# Autodesk Inventor assembly: Press
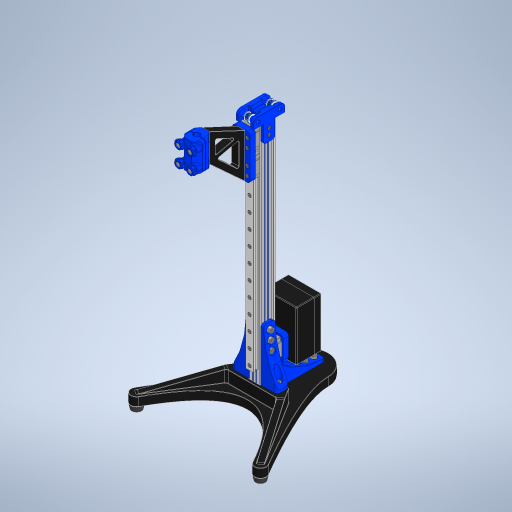
[picture p0: Inventor's stored thumbnail of the model, 512x512]
Saved by Autodesk Inventor 2024 (Build 280153000, 153)
## iProperties
Created: 2023-12-26
Part Number: Press
Document SubType Name: Assembly
Designer: denni
Author: denni
## Documents named in this file (28)
- D:\GIT\ThreadedInsertPress\Press.iam
- D:\GIT\ThreadedInsertPress\Parts\Others\AluminiumTSlotProfil20x20x420.ipt
- D:\GIT\ThreadedInsertPress\Parts\3D printed\PressBase.ipt
- D:\GIT\ThreadedInsertPress\Parts\Others\TS_04_12_364.ipt
- D:\Inventor\Content Center Files\R2024\de-DE\ISO 4762(1)\DIN EN ISO 4762 - M3 x 10.ipt
- D:\GIT\ThreadedInsertPress\Parts\3D printed\BraketBack.ipt
- D:\Inventor\Content Center Files\R2024\de-DE\ISO 4762(1)\DIN EN ISO 4762 - M5 x 16.ipt
- D:\Inventor\Content Center Files\R2024\de-DE\ISO 4762(1)\DIN EN ISO 4762 - M5 x 10.ipt
- D:\GIT\ThreadedInsertPress\Parts\3D printed\BraketSide.ipt
- D:\GIT\ThreadedInsertPress\Parts\Others\TW_04_12\TW_04_12.iam
- D:\GIT\ThreadedInsertPress\Parts\Others\RubberFeet\RubberFoot.iam
- D:\GIT\ThreadedInsertPress\Parts\3D printed\AdapterLinearGuideLong.ipt
- D:\Inventor\Content Center Files\R2024\de-DE\ISO 4762(1)\DIN EN ISO 4762 - M3 x 16.ipt
- D:\GIT\ThreadedInsertPress\Parts\3D printed\AdapterLinearGuideShort.ipt
- D:\GIT\ThreadedInsertPress\Parts\3D printed\IdlerBracket_Screws.ipt
- D:\GIT\ThreadedInsertPress\Parts\Others\Gt2TimingIdlerPulley16TW6B3\Gt2TimingIdlerPulley16TW6B3\Gt2TimingIdlerPulley16TW6B3.iam
- D:\GIT\ThreadedInsertPress\Parts\3D printed\IdlerBracket_Nuts.ipt
- D:\Inventor\Content Center Files\R2024\de-DE\ISO 4762(1)\DIN EN ISO 4762 - M3 x 6.ipt
- D:\Inventor\Content Center Files\R2024\de-DE\ISO 4762(1)\DIN EN ISO 4762 - M3 x 25.ipt
- D:\Inventor\Content Center Files\R2024\de-DE\ISO 4762(1)\DIN EN ISO 4762 - M5 x 20.ipt
- D:\GIT\ThreadedInsertPress\Parts\3D printed\ArmSolderingIron.ipt
- D:\GIT\ThreadedInsertPress\Parts\3D printed\BracketSolderingIron_1.ipt
- D:\Inventor\Content Center Files\R2024\de-DE\ISO 4762(1)\DIN EN ISO 4762 - M4 x 10.ipt
- D:\GIT\ThreadedInsertPress\Parts\3D printed\BracketSolderingIron_2.ipt
- D:\GIT\ThreadedInsertPress\Parts\3D printed\ScrewHead.ipt
- D:\Inventor\Content Center Files\R2024\de-DE\DIN EN ISO 4017\DIN EN ISO 4017 - M4 x 25.ipt
- D:\Inventor\Content Center Files\R2024\de-DE\DIN EN ISO 4032\DIN EN ISO 4032 - M3.ipt
- D:\GIT\ThreadedInsertPress\Parts\BatteryPack.iam
## Components (100 placed, 27 different names)
1. AluminiumTSlotProfil20x20x420:1 — Passend:1, Passend:2, Fluchtend:1, Fluchtend:2, Passend:3, Passend:4, Fluchtend:3, Fluchtend:4, Fluchtend:5, Passend:8, Passend:9, Fluchtend:6, Fluchtend:7, Passend:31, Passend:32, Passend:33, Fluchtend:8
2. PressBase:1 — Passend:1, Passend:2, Fluchtend:1, Passend:5, Passend:6, Passend:7, Passend:10, Passend:11, Passend:18, Passend:19, Passend:20, Passend:21, Passend:22, Passend:23
3. TS_04_12_364:1 — Fluchtend:2, Passend:3, Fluchtend:5, Einfügen:1, Einfügen:2, Einfügen:3, Einfügen:4, Einfügen:5, Einfügen:6, Einfügen:7, Einfügen:8, Einfügen:9, Einfügen:10, Einfügen:11, Einfügen:12, Einfügen:13, Einfügen:14, Einfügen:15, Passend:12, Passend:13, Passend:14, Passend:15
4. TS_04_12_364:2 — Passend:4, Fluchtend:3, Fluchtend:4, Einfügen:16, Einfügen:17, Einfügen:18, Einfügen:19, Einfügen:20, Einfügen:21, Einfügen:22, Einfügen:23, Einfügen:24, Einfügen:25, Einfügen:26, Einfügen:27, Einfügen:28, Einfügen:29, Einfügen:30, Passend:16, Passend:17
5. DIN EN ISO 4762 M3 x 10:1 — Einfügen:1
6. DIN EN ISO 4762 M3 x 10:2 — Einfügen:2
7. DIN EN ISO 4762 M3 x 10:3 — Einfügen:3
8. DIN EN ISO 4762 M3 x 10:4 — Einfügen:4
9. DIN EN ISO 4762 M3 x 10:5 — Einfügen:5
10. DIN EN ISO 4762 M3 x 10:6 — Einfügen:6
11. DIN EN ISO 4762 M3 x 10:7 — Einfügen:7
12. DIN EN ISO 4762 M3 x 10:8 — Einfügen:8
13. DIN EN ISO 4762 M3 x 10:9 — Einfügen:9
14. DIN EN ISO 4762 M3 x 10:10 — Einfügen:10
15. DIN EN ISO 4762 M3 x 10:11 — Einfügen:11
16. DIN EN ISO 4762 M3 x 10:12 — Einfügen:12
17. DIN EN ISO 4762 M3 x 10:13 — Einfügen:13
18. DIN EN ISO 4762 M3 x 10:14 — Einfügen:14
19. DIN EN ISO 4762 M3 x 10:15 — Einfügen:15
20. DIN EN ISO 4762 M3 x 10:16 — Einfügen:16
21. DIN EN ISO 4762 M3 x 10:17 — Einfügen:17
22. DIN EN ISO 4762 M3 x 10:18 — Einfügen:18
23. DIN EN ISO 4762 M3 x 10:19 — Einfügen:19
24. DIN EN ISO 4762 M3 x 10:20 — Einfügen:20
25. DIN EN ISO 4762 M3 x 10:21 — Einfügen:21
26. DIN EN ISO 4762 M3 x 10:22 — Einfügen:22
27. DIN EN ISO 4762 M3 x 10:23 — Einfügen:23
28. DIN EN ISO 4762 M3 x 10:24 — Einfügen:24
29. DIN EN ISO 4762 M3 x 10:25 — Einfügen:25
30. DIN EN ISO 4762 M3 x 10:26 — Einfügen:26
31. DIN EN ISO 4762 M3 x 10:27 — Einfügen:27
32. DIN EN ISO 4762 M3 x 10:28 — Einfügen:28
33. DIN EN ISO 4762 M3 x 10:29 — Einfügen:29
34. DIN EN ISO 4762 M3 x 10:30 — Einfügen:30
35. BraketBack:1 — Passend:5, Passend:6, Passend:7, Einfügen:31, Einfügen:32, Einfügen:33, Einfügen:34, Einfügen:35
36. DIN EN ISO 4762 M5 x 16:1 — Einfügen:31
37. DIN EN ISO 4762 M5 x 16:2 — Einfügen:32
38. DIN EN ISO 4762 M5 x 16:3 — Einfügen:33
39. DIN EN ISO 4762 M5 x 10:1 — Einfügen:34
40. DIN EN ISO 4762 M5 x 10:2 — Einfügen:35
41. BraketSide:1 — Passend:9, Passend:10, Fluchtend:6, Einfügen:36, Einfügen:37, Einfügen:38, Einfügen:39
42. BraketSide:2 — Passend:8, Passend:11, Fluchtend:7, Einfügen:40, Einfügen:41, Einfügen:42, Einfügen:43
43. DIN EN ISO 4762 M5 x 16:4 — Einfügen:36
44. DIN EN ISO 4762 M5 x 10:3 — Einfügen:37
45. DIN EN ISO 4762 M5 x 10:4 — Einfügen:38
46. DIN EN ISO 4762 M5 x 10:5 — Einfügen:39
47. DIN EN ISO 4762 M5 x 10:6 — Einfügen:40
48. DIN EN ISO 4762 M5 x 10:7 — Einfügen:41
49. DIN EN ISO 4762 M5 x 10:8 — Einfügen:42
50. DIN EN ISO 4762 M5 x 16:5 — Einfügen:43
51. TW_04_12:1 [sub-assembly] — Passend:13, Passend:15, Passend:24, Passend:25, Passend:26
52. TW_04_12:2 [sub-assembly] — Passend:12, Passend:14, Passend:24, Passend:27
53. TW_04_12:3 [sub-assembly] — Passend:16, Passend:17, Passend:28, Passend:29, Passend:30
54. RubberFoot:1 [sub-assembly] — Passend:18, Passend:22
55. RubberFoot:2 [sub-assembly] — Passend:19, Passend:21
56. RubberFoot:3 [sub-assembly] — Passend:20, Passend:23
57. AdapterLinearGuideLong:1 — Passend:25, Passend:26, Passend:27, Einfügen:44, Einfügen:45, Einfügen:46, Einfügen:47, Einfügen:48, Einfügen:49, Einfügen:50, Einfügen:51, Passend:39, Passend:40, Passend:41, Einfügen:63, Einfügen:64, Einfügen:65
58. DIN EN ISO 4762 M3 x 16:1 — Einfügen:44
59. DIN EN ISO 4762 M3 x 16:2 — Einfügen:45
60. DIN EN ISO 4762 M3 x 16:3 — Einfügen:46
61. DIN EN ISO 4762 M3 x 16:4 — Einfügen:47
62. DIN EN ISO 4762 M3 x 16:5 — Einfügen:48
63. DIN EN ISO 4762 M3 x 16:6 — Einfügen:49
64. DIN EN ISO 4762 M3 x 16:7 — Einfügen:50
65. DIN EN ISO 4762 M3 x 16:8 — Einfügen:51
66. AdapterLinearGuideShort:1 — Passend:28, Einfügen:52, Einfügen:53, Einfügen:54, Einfügen:55, Passend:29, Passend:30, Passend:58, Passend:59, Passend:60
67. DIN EN ISO 4762 M3 x 16:9 — Einfügen:52
68. DIN EN ISO 4762 M3 x 16:10 — Einfügen:53
69. DIN EN ISO 4762 M3 x 16:11 — Einfügen:54
70. DIN EN ISO 4762 M3 x 16:12 — Einfügen:55
71. IdlerBracket_Screws:1 — Passend:31, Passend:32, Passend:33, Passend:34, Passend:35, Passend:36, Passend:37, Fluchtend:9, Passend:38, Einfügen:56, Einfügen:57, Einfügen:58, Einfügen:59, Einfügen:60
72. Gt2TimingIdlerPulley16TW6B3:1 [sub-assembly] — Passend:34, Passend:37
73. Gt2TimingIdlerPulley16TW6B3:2 [sub-assembly] — Passend:35, Passend:36
74. IdlerBracket_Nuts:1 — Fluchtend:8, Fluchtend:9, Passend:38, Einfügen:61, Einfügen:62, Einfügen:72, Einfügen:73
75. DIN EN ISO 4762 M3 x 6:1 — Einfügen:56
76. DIN EN ISO 4762 M3 x 6:2 — Einfügen:57
77. DIN EN ISO 4762 M3 x 25:1 — Einfügen:58
78. DIN EN ISO 4762 M3 x 25:2 — Einfügen:59
79. DIN EN ISO 4762 M5 x 20:1 — Einfügen:60
80. DIN EN ISO 4762 M3 x 6:3 — Einfügen:61
81. DIN EN ISO 4762 M3 x 6:4 — Einfügen:62
82. ArmSolderingIron:1 — Passend:39, Passend:40, Passend:41, Passend:43, Passend:44, Passend:45
83. DIN EN ISO 4762 M5 x 10:9 — Einfügen:63
84. DIN EN ISO 4762 M5 x 10:10 — Einfügen:64
85. DIN EN ISO 4762 M5 x 10:11 — Einfügen:65
86. BracketSolderingIron_1:1 — Passend:43, Einfügen:66, Einfügen:67, Passend:44, Passend:45, Passend:46, Passend:47, Passend:57
87. DIN EN ISO 4762 M4 x 10:1 — Einfügen:66
88. DIN EN ISO 4762 M4 x 10:2 — Einfügen:67
89. BracketSolderingIron_2:1 — Passend:46, Passend:47, Passend:49, Passend:50, Passend:51, Passend:52, Passend:53, Passend:54, Passend:55, Passend:56, Passend:57
90. ScrewHead:1 — Passend:50, Passend:53, Fluchtend:10, Einfügen:68
91. ScrewHead:2 — Passend:52, Passend:56, Fluchtend:11, Einfügen:71
92. ScrewHead:3 — Passend:51, Passend:54, Fluchtend:11, Einfügen:70
93. ScrewHead:4 — Passend:49, Passend:55, Fluchtend:10, Einfügen:69
94. DIN EN ISO 4017 M4 x 25:1 — Einfügen:68
95. DIN EN ISO 4017 M4 x 25:2 — Einfügen:69
96. DIN EN ISO 4017 M4 x 25:3 — Einfügen:70
97. DIN EN ISO 4017 M4 x 25:4 — Einfügen:71
98. DIN EN ISO 4032 M3:1 — Einfügen:72, Fluchtend:12
99. DIN EN ISO 4032 M3:2 — Einfügen:73, Fluchtend:12
100. BatteryPack:1 [sub-assembly] — Passend:58, Passend:59, Passend:60
## Relationships (143: Insert 73, Mate 58, Flush 12)
- Passend:1 [Mate]: AluminiumTSlotProfil20x20x420:1 ↔ PressBase:1
- Passend:2 [Mate]: AluminiumTSlotProfil20x20x420:1 ↔ PressBase:1
- Fluchtend:1 [Flush]: AluminiumTSlotProfil20x20x420:1 ↔ PressBase:1
- Fluchtend:2 [Flush] (-4 mm): AluminiumTSlotProfil20x20x420:1 ↔ TS_04_12_364:1
- Passend:3 [Mate]: AluminiumTSlotProfil20x20x420:1 ↔ TS_04_12_364:1
- Passend:4 [Mate]: AluminiumTSlotProfil20x20x420:1 ↔ TS_04_12_364:2
- Fluchtend:3 [Flush] (4 mm): AluminiumTSlotProfil20x20x420:1 ↔ TS_04_12_364:2
- Fluchtend:4 [Flush]: AluminiumTSlotProfil20x20x420:1 ↔ TS_04_12_364:2
- Fluchtend:5 [Flush]: AluminiumTSlotProfil20x20x420:1 ↔ TS_04_12_364:1
- Einfügen:1 [Insert]: TS_04_12_364:1 ↔ DIN EN ISO 4762 M3 x 10:1
- Einfügen:2 [Insert]: TS_04_12_364:1 ↔ DIN EN ISO 4762 M3 x 10:2
- Einfügen:3 [Insert]: TS_04_12_364:1 ↔ DIN EN ISO 4762 M3 x 10:3
- Einfügen:4 [Insert]: TS_04_12_364:1 ↔ DIN EN ISO 4762 M3 x 10:4
- Einfügen:5 [Insert]: TS_04_12_364:1 ↔ DIN EN ISO 4762 M3 x 10:5
- Einfügen:6 [Insert]: TS_04_12_364:1 ↔ DIN EN ISO 4762 M3 x 10:6
- Einfügen:7 [Insert]: TS_04_12_364:1 ↔ DIN EN ISO 4762 M3 x 10:7
- Einfügen:8 [Insert]: TS_04_12_364:1 ↔ DIN EN ISO 4762 M3 x 10:8
- Einfügen:9 [Insert]: TS_04_12_364:1 ↔ DIN EN ISO 4762 M3 x 10:9
- Einfügen:10 [Insert]: TS_04_12_364:1 ↔ DIN EN ISO 4762 M3 x 10:10
- Einfügen:11 [Insert]: TS_04_12_364:1 ↔ DIN EN ISO 4762 M3 x 10:11
- Einfügen:12 [Insert]: TS_04_12_364:1 ↔ DIN EN ISO 4762 M3 x 10:12
- Einfügen:13 [Insert]: TS_04_12_364:1 ↔ DIN EN ISO 4762 M3 x 10:13
- Einfügen:14 [Insert]: TS_04_12_364:1 ↔ DIN EN ISO 4762 M3 x 10:14
- Einfügen:15 [Insert]: TS_04_12_364:1 ↔ DIN EN ISO 4762 M3 x 10:15
- Einfügen:16 [Insert]: TS_04_12_364:2 ↔ DIN EN ISO 4762 M3 x 10:16
- Einfügen:17 [Insert]: TS_04_12_364:2 ↔ DIN EN ISO 4762 M3 x 10:17
- Einfügen:18 [Insert]: TS_04_12_364:2 ↔ DIN EN ISO 4762 M3 x 10:18
- Einfügen:19 [Insert]: TS_04_12_364:2 ↔ DIN EN ISO 4762 M3 x 10:19
- Einfügen:20 [Insert]: TS_04_12_364:2 ↔ DIN EN ISO 4762 M3 x 10:20
- Einfügen:21 [Insert]: TS_04_12_364:2 ↔ DIN EN ISO 4762 M3 x 10:21
- Einfügen:22 [Insert]: TS_04_12_364:2 ↔ DIN EN ISO 4762 M3 x 10:22
- Einfügen:23 [Insert]: TS_04_12_364:2 ↔ DIN EN ISO 4762 M3 x 10:23
- Einfügen:24 [Insert]: TS_04_12_364:2 ↔ DIN EN ISO 4762 M3 x 10:24
- Einfügen:25 [Insert]: TS_04_12_364:2 ↔ DIN EN ISO 4762 M3 x 10:25
- Einfügen:26 [Insert]: TS_04_12_364:2 ↔ DIN EN ISO 4762 M3 x 10:26
- Einfügen:27 [Insert]: TS_04_12_364:2 ↔ DIN EN ISO 4762 M3 x 10:27
- Einfügen:28 [Insert]: TS_04_12_364:2 ↔ DIN EN ISO 4762 M3 x 10:28
- Einfügen:29 [Insert]: TS_04_12_364:2 ↔ DIN EN ISO 4762 M3 x 10:29
- Einfügen:30 [Insert]: TS_04_12_364:2 ↔ DIN EN ISO 4762 M3 x 10:30
- Passend:5 [Mate]: PressBase:1 ↔ BraketBack:1
- Passend:6 [Mate]: PressBase:1 ↔ BraketBack:1
- Passend:7 [Mate]: PressBase:1 ↔ BraketBack:1
- Einfügen:31 [Insert]: BraketBack:1 ↔ DIN EN ISO 4762 M5 x 16:1
- Einfügen:32 [Insert]: BraketBack:1 ↔ DIN EN ISO 4762 M5 x 16:2
- Einfügen:33 [Insert]: BraketBack:1 ↔ DIN EN ISO 4762 M5 x 16:3
- Einfügen:34 [Insert]: BraketBack:1 ↔ DIN EN ISO 4762 M5 x 10:1
- Einfügen:35 [Insert]: BraketBack:1 ↔ DIN EN ISO 4762 M5 x 10:2
- Passend:8 [Mate]: AluminiumTSlotProfil20x20x420:1 ↔ BraketSide:2
- Passend:9 [Mate]: AluminiumTSlotProfil20x20x420:1 ↔ BraketSide:1
- Passend:10 [Mate]: PressBase:1 ↔ BraketSide:1
- Passend:11 [Mate]: PressBase:1 ↔ BraketSide:2
- Fluchtend:6 [Flush]: AluminiumTSlotProfil20x20x420:1 ↔ BraketSide:1
- Fluchtend:7 [Flush]: AluminiumTSlotProfil20x20x420:1 ↔ BraketSide:2
- Einfügen:36 [Insert]: BraketSide:1 ↔ DIN EN ISO 4762 M5 x 16:4
- Einfügen:37 [Insert]: BraketSide:1 ↔ DIN EN ISO 4762 M5 x 10:3
- Einfügen:38 [Insert]: BraketSide:1 ↔ DIN EN ISO 4762 M5 x 10:4
- Einfügen:39 [Insert]: BraketSide:1 ↔ DIN EN ISO 4762 M5 x 10:5
- Einfügen:40 [Insert]: BraketSide:2 ↔ DIN EN ISO 4762 M5 x 10:6
- Einfügen:41 [Insert]: BraketSide:2 ↔ DIN EN ISO 4762 M5 x 10:7
- Einfügen:42 [Insert]: BraketSide:2 ↔ DIN EN ISO 4762 M5 x 10:8
- Einfügen:43 [Insert]: BraketSide:2 ↔ DIN EN ISO 4762 M5 x 16:5
- Passend:12 [Mate]: TS_04_12_364:1 ↔ TW_04_12:2
- Passend:13 [Mate]: TS_04_12_364:1 ↔ TW_04_12:1
- Passend:14 [Mate]: TS_04_12_364:1 ↔ TW_04_12:2
- Passend:15 [Mate]: TS_04_12_364:1 ↔ TW_04_12:1
- Passend:16 [Mate]: TS_04_12_364:2 ↔ TW_04_12:3
- Passend:17 [Mate]: TS_04_12_364:2 ↔ TW_04_12:3
- Passend:18 [Mate]: PressBase:1 ↔ RubberFoot:1
- Passend:19 [Mate]: PressBase:1 ↔ RubberFoot:2
- Passend:20 [Mate]: PressBase:1 ↔ RubberFoot:3
- Passend:21 [Mate]: PressBase:1 ↔ RubberFoot:2
- Passend:22 [Mate]: PressBase:1 ↔ RubberFoot:1
- Passend:23 [Mate]: PressBase:1 ↔ RubberFoot:3
- Passend:24 [Mate] (-75 mm): TW_04_12:1 ↔ TW_04_12:2
- Passend:25 [Mate]: TW_04_12:1 ↔ AdapterLinearGuideLong:1
- Passend:26 [Mate]: TW_04_12:1 ↔ AdapterLinearGuideLong:1
- Passend:27 [Mate]: TW_04_12:2 ↔ AdapterLinearGuideLong:1
- Einfügen:44 [Insert]: AdapterLinearGuideLong:1 ↔ DIN EN ISO 4762 M3 x 16:1
- Einfügen:45 [Insert]: AdapterLinearGuideLong:1 ↔ DIN EN ISO 4762 M3 x 16:2
- Einfügen:46 [Insert]: AdapterLinearGuideLong:1 ↔ DIN EN ISO 4762 M3 x 16:3
- Einfügen:47 [Insert]: AdapterLinearGuideLong:1 ↔ DIN EN ISO 4762 M3 x 16:4
- Einfügen:48 [Insert]: AdapterLinearGuideLong:1 ↔ DIN EN ISO 4762 M3 x 16:5
- Einfügen:49 [Insert]: AdapterLinearGuideLong:1 ↔ DIN EN ISO 4762 M3 x 16:6
- Einfügen:50 [Insert]: AdapterLinearGuideLong:1 ↔ DIN EN ISO 4762 M3 x 16:7
- Einfügen:51 [Insert]: AdapterLinearGuideLong:1 ↔ DIN EN ISO 4762 M3 x 16:8
- Passend:28 [Mate]: TW_04_12:3 ↔ AdapterLinearGuideShort:1
- Einfügen:52 [Insert]: AdapterLinearGuideShort:1 ↔ DIN EN ISO 4762 M3 x 16:9
- Einfügen:53 [Insert]: AdapterLinearGuideShort:1 ↔ DIN EN ISO 4762 M3 x 16:10
- Einfügen:54 [Insert]: AdapterLinearGuideShort:1 ↔ DIN EN ISO 4762 M3 x 16:11
- Einfügen:55 [Insert]: AdapterLinearGuideShort:1 ↔ DIN EN ISO 4762 M3 x 16:12
- Passend:29 [Mate]: TW_04_12:3 ↔ AdapterLinearGuideShort:1
- Passend:30 [Mate]: TW_04_12:3 ↔ AdapterLinearGuideShort:1
- Passend:31 [Mate]: AluminiumTSlotProfil20x20x420:1 ↔ IdlerBracket_Screws:1
- Passend:32 [Mate]: AluminiumTSlotProfil20x20x420:1 ↔ IdlerBracket_Screws:1
- Passend:33 [Mate]: AluminiumTSlotProfil20x20x420:1 ↔ IdlerBracket_Screws:1
- Passend:34 [Mate]: IdlerBracket_Screws:1 ↔ Gt2TimingIdlerPulley16TW6B3:1
- Passend:35 [Mate]: IdlerBracket_Screws:1 ↔ Gt2TimingIdlerPulley16TW6B3:2
- Passend:36 [Mate] (0.5 mm): IdlerBracket_Screws:1 ↔ Gt2TimingIdlerPulley16TW6B3:2
- Passend:37 [Mate] (0.5 mm): IdlerBracket_Screws:1 ↔ Gt2TimingIdlerPulley16TW6B3:1
- Fluchtend:8 [Flush]: AluminiumTSlotProfil20x20x420:1 ↔ IdlerBracket_Nuts:1
- Fluchtend:9 [Flush]: IdlerBracket_Screws:1 ↔ IdlerBracket_Nuts:1
- Passend:38 [Mate]: IdlerBracket_Screws:1 ↔ IdlerBracket_Nuts:1
- Einfügen:56 [Insert]: IdlerBracket_Screws:1 ↔ DIN EN ISO 4762 M3 x 6:1
- Einfügen:57 [Insert]: IdlerBracket_Screws:1 ↔ DIN EN ISO 4762 M3 x 6:2
- Einfügen:58 [Insert]: IdlerBracket_Screws:1 ↔ DIN EN ISO 4762 M3 x 25:1
- Einfügen:59 [Insert]: IdlerBracket_Screws:1 ↔ DIN EN ISO 4762 M3 x 25:2
- Einfügen:60 [Insert]: IdlerBracket_Screws:1 ↔ DIN EN ISO 4762 M5 x 20:1
- Einfügen:61 [Insert]: IdlerBracket_Nuts:1 ↔ DIN EN ISO 4762 M3 x 6:3
- Einfügen:62 [Insert]: IdlerBracket_Nuts:1 ↔ DIN EN ISO 4762 M3 x 6:4
- Passend:39 [Mate]: AdapterLinearGuideLong:1 ↔ ArmSolderingIron:1
- Passend:40 [Mate]: AdapterLinearGuideLong:1 ↔ ArmSolderingIron:1
- Passend:41 [Mate]: AdapterLinearGuideLong:1 ↔ ArmSolderingIron:1
- Einfügen:63 [Insert]: AdapterLinearGuideLong:1 ↔ DIN EN ISO 4762 M5 x 10:9
- Einfügen:64 [Insert]: AdapterLinearGuideLong:1 ↔ DIN EN ISO 4762 M5 x 10:10
- Einfügen:65 [Insert]: AdapterLinearGuideLong:1 ↔ DIN EN ISO 4762 M5 x 10:11
- Passend:43 [Mate]: ArmSolderingIron:1 ↔ BracketSolderingIron_1:1
- Einfügen:66 [Insert]: BracketSolderingIron_1:1 ↔ DIN EN ISO 4762 M4 x 10:1
- Einfügen:67 [Insert]: BracketSolderingIron_1:1 ↔ DIN EN ISO 4762 M4 x 10:2
- Passend:44 [Mate]: ArmSolderingIron:1 ↔ BracketSolderingIron_1:1
- Passend:45 [Mate]: ArmSolderingIron:1 ↔ BracketSolderingIron_1:1
- Passend:46 [Mate]: BracketSolderingIron_1:1 ↔ BracketSolderingIron_2:1
- Passend:47 [Mate]: BracketSolderingIron_1:1 ↔ BracketSolderingIron_2:1
- Passend:49 [Mate]: BracketSolderingIron_2:1 ↔ ScrewHead:4
- Passend:50 [Mate]: BracketSolderingIron_2:1 ↔ ScrewHead:1
- Passend:51 [Mate]: BracketSolderingIron_2:1 ↔ ScrewHead:3
- Passend:52 [Mate]: BracketSolderingIron_2:1 ↔ ScrewHead:2
- Passend:53 [Mate]: BracketSolderingIron_2:1 ↔ ScrewHead:1
- Passend:54 [Mate]: BracketSolderingIron_2:1 ↔ ScrewHead:3
- Passend:55 [Mate]: BracketSolderingIron_2:1 ↔ ScrewHead:4
- Passend:56 [Mate]: BracketSolderingIron_2:1 ↔ ScrewHead:2
- Fluchtend:10 [Flush]: ScrewHead:1 ↔ ScrewHead:4
- Fluchtend:11 [Flush]: ScrewHead:2 ↔ ScrewHead:3
- Einfügen:68 [Insert]: ScrewHead:1 ↔ DIN EN ISO 4017 M4 x 25:1
- Einfügen:69 [Insert]: ScrewHead:4 ↔ DIN EN ISO 4017 M4 x 25:2
- Einfügen:70 [Insert]: ScrewHead:3 ↔ DIN EN ISO 4017 M4 x 25:3
- Einfügen:71 [Insert]: ScrewHead:2 ↔ DIN EN ISO 4017 M4 x 25:4
- Einfügen:72 [Insert]: IdlerBracket_Nuts:1 ↔ DIN EN ISO 4032 M3:1
- Einfügen:73 [Insert]: IdlerBracket_Nuts:1 ↔ DIN EN ISO 4032 M3:2
- Fluchtend:12 [Flush]: DIN EN ISO 4032 M3:1 ↔ DIN EN ISO 4032 M3:2
- Passend:57 [Mate]: BracketSolderingIron_1:1 ↔ BracketSolderingIron_2:1
- Passend:58 [Mate]: AdapterLinearGuideShort:1 ↔ BatteryPack:1
- Passend:59 [Mate]: AdapterLinearGuideShort:1 ↔ BatteryPack:1
- Passend:60 [Mate]: AdapterLinearGuideShort:1 ↔ BatteryPack:1
